# Autodesk Inventor assembly: Receiver
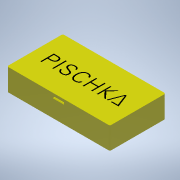
[picture p0: Inventor's stored thumbnail of the model, 180x180]
Saved by Autodesk Inventor 2020.1 (Build 241239000, 239)
## iProperties
Created: 2019-07-14
Part Number: Receiver
Document SubType Name: Assembly
Designer: Petar
Author: Petar
## Documents named in this file (10)
- D:\OMG\E-Board\CAD\Inventor\Remote\Receiver.iam
- D:\OMG\E-Board\CAD\Inventor\Remote\Receiver Case.ipt
- D:\OMG\E-Board\CAD\Inventor\Electrical Components\nRF24L01+_enhanced.ipt
- D:\OMG\E-Board\CAD\Inventor\Electrical Components\Arduino Nano\arduino nano.iam
- D:\OMG\E-Board\CAD\Inventor\Electrical Components\Cirquit Parts\PushBtn.ipt
- D:\OMG\E-Board\CAD\Inventor\Electrical Components\Cirquit Parts\LED-Diode bent 5mm.iam
- D:\OMG\E-Board\CAD\Inventor\Electrical Components\HM-10 Bluetooth 4.0 BLE Module.ipt
- D:\OMG\E-Board\CAD\Inventor\Electrical Components\Cirquit Parts\DS1071-1xN (BLS)\DS1071-1x5.ipt
- D:\OMG\E-Board\CAD\Inventor\Remote\Receiver Lid.ipt
- D:\OMG\E-Board\CAD\Inventor\Electrical Components\Receiver Pins.iam
## Components (9 placed, 9 different names)
1. Receiver Case:1 — Rigid:1, Rigid:3, Rigid:10, Rigid:11, Rigid:12, Rigid:13, Rigid:14
2. nRF24L01+_enhanced:1 — Rigid:13
3. arduino nano:1 [sub-assembly] — Rigid:1
4. PushBtn:1 — Rigid:11
5. LED-Diode bent 5mm:1 [sub-assembly] — Rigid:3
6. HM-10 Bluetooth 4.0 BLE Module:1 — Rigid:6, Rigid:12
7. DS1071-1x5:1 — Rigid:6
8. Receiver Pins:1 [sub-assembly] — Rigid:14
9. Receiver Lid:1 — Rigid:10
## Relationships (8: WeldJoint 8)
- Rigid:1 [WeldJoint]: Receiver Case:1 ↔ arduino nano:1
- Rigid:3 [WeldJoint] (1.75 mm): Receiver Case:1 ↔ LED-Diode bent 5mm:1
- Rigid:6 [WeldJoint] (2.5 mm): HM-10 Bluetooth 4.0 BLE Module:1 ↔ DS1071-1x5:1
- Rigid:10 [WeldJoint]: Receiver Case:1 ↔ Receiver Lid:1
- Rigid:11 [WeldJoint]: Receiver Case:1 ↔ PushBtn:1
- Rigid:12 [WeldJoint]: Receiver Case:1 ↔ HM-10 Bluetooth 4.0 BLE Module:1
- Rigid:13 [WeldJoint]: Receiver Case:1 ↔ nRF24L01+_enhanced:1
- Rigid:14 [WeldJoint]: Receiver Case:1 ↔ Receiver Pins:1
